# Autodesk Inventor assembly: 048-DXP(R,D-129)(F,D-166-3)
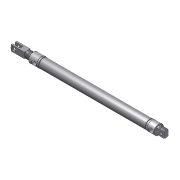
[picture p0: Inventor's stored thumbnail of the model, 180x180]
Saved by Autodesk Inventor 2012 (Build 160160000, 160)
## iProperties
Category: PARTsolutions
Created: 2013-01-19
Part Number: 048-DXP(R,D-129)(F,D-166-3)
Catalog Web Link: www.cadenas.de
Description: Original Line Standard Air Cylinders -
Document SubType Name: Assembly
Designer: PARTsolutions
NB: 048-DXP(R,D-129)(F,D-166-3)
NN: Original Line Standard Air Cylinders
NBSYN: $PNC.
LINA: 048-DXP
PSOL_MULTISOLIDPART: 0.0
PN: 048-DXP
PNC: 048-DXP(R,D-129)(F,D-166-3)
PNA: (D-129)(D-166-3)
DASH: -
BORE1: 0.75000000
BORE: 3/4" (04)
BOREPN: 04
STROKE: 8.000
STROKEALG: [0.011:50/0.001]
STROKE1: 8.000
ACTING: D
ACTINGALG: '' , 'Single Acting (SA)' , 'R' , 'Reverse Single Acting (SA)' , 'D' , 'Double Acting (SA)'
ACTINGPN: D
MNT: XP
MNTALG: '' , 'Front Nose Mounting (SA)' , 'P' , 'Rear Pivot Mounting (SA)' , 'XP' , 'Double End or Pivot Mounting (SA)' , 'X' , 'Double End Mounting (SA)' , 'BF' , 'Front Block Mounting (SA)' , 'BR' , 'Rear Block Mounting for Vertical Positioning (SA)' , 'BFT' , 'Front Block Trunnion Mounting (SA)' , 'BRT' , 'Rear Block Trunnion Mounting (SA)'
MNTPN: XP
DERALG: '' , 'N/A'
NRALG: '' , 'N/A'
BMALG: '' , 'N/A'
COALG: '' , 'N/A'
OOALG: '', 'N/A'
VO: Z
VOALG: 'Z' , 'N/A'
MALG: '', 'Without Magnet', 'M', 'With Magnet'
EEL: 0.000
EEMAX: 42.0000
EEALG: '', 'Without Extra Extension', 'EE', 'With Extra Extension'
EELALG: 0
EEPN1: 0.000
KALG: '', 'Standard' , 'K' , 'Ports Rotated 90deg K'
QALG: '' , 'N/A'
YALG: '' , 'Without Pivot Bushing' , 'Y' , 'With Pivot Bushing'
FALG: '', 'Non-Coated (Standard)', 'F', 'Molycoated'
TALG: '' , 'Standard -20° to 200°F (-29° to 95°C)' , 'N' , 'Low Temperature' , 'V' , 'High Temperature'
BALG: '', 'W/out Bumpers' , 'B' , 'W/ Bumpers'
HALG: '', 'N/A'
SERALG: '' , 'Without Spring Extend/Return' , 'JS' , 'With Spring Return' , 'JR' , 'With Spring Extend'
SRALG: '' , 'Standard Stainless Steel'
SRCON: 0
WALG: '' , 'Without Wiper' , 'W' , 'With Wiper'
EALG: '' , 'Standard Seals/Lube' , 'E' , 'Non-Lube Seals/Lube'
HLALG: '' , 'Without Low Pressure Hydraulic' , 'HL' , 'With Low Pressure Hydraulic'
STALG: '' , 'N/A'
STPT1ALG: '' , 'N/A'
STPT2ALG: '' , 'N/A'
STPT3ALG: '' , 'N/A'
STPT4ALG: '' , 'N/A'
MB: R,D-129
MBALG: '' , 'Without Mounting Bracket' , 'F,D-129' , 'D-129 (front)'  , 'R,D-129' , 'D-129 (rear)' , '2x,D-129' , 'D-129 (front & rear)'
MBPN: (R,D-129)
MBPNALL: D-129
MBPNALLREAR: D-129
PBALG: '' , 'N/A'
PBPNALL: D-13498-A
PRC: F,D-166-3
PRCALG: '' , 'W/out Pivot Rod Clevis' , 'F,D-166-3' , 'D-166-3 (front)'
PRCPN: (F,D-166-3)
PRCPNALL: D-166-3
TBALG: '' , 'N/A'
MNALG: '' , 'N/A'
TLEN: 9.2555
FRAC: 74.7500
RGDACCON: R
RHCON: P
RHCON1: P
RHCONON: 1
FNUTCON: 1
RNUTCON: 1
FNUTPN: D-9
RNUTPN: D-9
FNUTTRANS: 0.0000
RNUTTRANS: 0.0000
VHOLECON: 0
A1: 1.5940
A1N: 0.8750
A1P: 1.5940
A1B: 1.5940
A4: 0.2525
A4N: 0.3130
A4P: 0.2525
A5: 0.0300
A1H: 1.594
A1NH: 0.5310
A1PH: 1.5940
A1BH: 1.0940
A1SH: 1.2190
A2H: 0.2190
A2NH: 0.2190
LENGTH: 3.7500
LENGTH1: 3.7500
LENGTH2: 3.8100
MUL: 8.0000
MUL11: 8.0000
MUL22: 21.520
MUL33: 13.5200
MUL2: 8.0000
MUL211: 8.0000
MUL222: 2.6900
MUL233: 1.6900
SSS: 16.0000
RGLEN: 1.3715
RHLEN: 1.1230
SSS1: 9.0000
A13: 1.3120
DIF: 0.0000
G5: 0.6250
ON: 0
SSADD: 0.0000
BADD: 0.0000
MADD: 0.0000
NVADD: 0.0000
TRACKL: 8.9655
TRACKCON: D-74168
TRIMCON: 0
TRIMCON1: 0
PINCON: D-51
FSPACE: 0.8211
SPACE: 0.1286
TEXT: 0.2250
S1: 1.0000
D1: 0.8325
D1N: 0.8050
D1B: 0.8625
D1P: 0.8325
FA: 0.940
RA: 0.9400
PPATH: standard_air_cylinder_asmtpl.prj
MATALGHTML: <b>Standard Original Line:</b><dl><dt>Rod:</dt><dd>- Stainless Steel</dd><dd>&nbsp;&nbsp;(5/16 ? 9/16 Bores)</dd><dd>- High Strength Carbon Steel</dd><dd>&nbsp;&nbsp;(3/4 ? 3 Bore)</dd><dd>- Stainless Steel</dd><dd>&nbsp;&nbsp;(?X? style DXP/DX/DXDE?)</dd><dt>Bearings:</dt><dd>- Sintered Bronze</dd><dt>Body:</dt><dd>- 304 Stainless Steel</dd><dt>End Caps:</dt><dd>- Aluminum</dd><dt>Seals:</dt><dd>- Buna N</dd></dl>
ASSCFGPRA: 04DXP
MBPNA: (D-129)
PRCPNA: (D-166-3)
ASSOPTACC: STPT4
A: 11.75
HADD: 0.0000
WFL: 0.250
QADD: 0.000
QADD1: 0.440
TEST: 8.0000
STDNUTF: 1
STDNUTR: 1
KT: DUMMY
CreationOption_UseAsmMates: false
SUPPLIER: Bimba
ARTICLENO: 048-DXP(R,D-129)(F,D-166-3)
BOMINFO: 048-DXP
CREATOR: CADENAS GmbH
PSOL_IDENT_0: {\\10.0.0.242\data_v9\23d-libs\bimba\bimba\bimba_imperial\bimba_full_line\original_line_cylinders\st
PSOL_IDENT_1: andard_air_cylinders\standard_air_cylinder_asmtab.prj},325 {VTYP=3D},{STYP=ASSTAB},{NB=048-DXP(R,D-1
PSOL_IDENT_2: 29)(F,D-166-3)},{LINA=048-DXP},{NN=Original Line Standard Air Cylinders},{DATE=06.09.2012 11:26:56},
PSOL_IDENT_3: {GEOMDATE=06.09.2012},{VERSION=},{LINEID=50},{LINESUBID=-1},{WBVAR=STROKE,ACTING,MNT,DER,NR,BM,CO,OO
PSOL_IDENT_4: ,VO,M,EE,EEL,K,Q,Y,G,T,B,H,SER,SR,NT,W,HL,STPT1,STPT2,STPT3,STPT4,MB,PB,PRC,TB,MN}  {NB=048-DXP(R,D-
PSOL_IDENT_5: 129)(F,D-166-3)},{LINA=048-DXP},{KT=DUMMY},{PN=048-DXP},{PNC=048-DXP(R,D-129)(F,D-166-3)},{PNA=(D-12
PSOL_IDENT_6: 9)(D-166-3)},{DASH=-},{BORE1=0.75000000},{BORE=3/4\" (04)},{BOREPN=04},{STROKE=8.000},{STROKEALG=[0.
PSOL_IDENT_7: 011:50/0.001]},{STROKE1=8.000},{ACTING=D},{ACTINGALG= '' , 'Single Acting (SA)' , 'R' , 'Reverse Sin
PSOL_IDENT_8: gle Acting (SA)' , 'D' , 'Double Acting (SA)' },{ACTINGPN=D},{MNT=XP},{MNTALG= '' , 'Front Nose Moun
PSOL_IDENT_9: ting (SA)' , 'P' , 'Rear Pivot Mounting (SA)' , 'XP' , 'Double End or Pivot Mounting (SA)' , 'X' , '
PSOL_IDENT_10: Double End Mounting (SA)' , 'BF' , 'Front Block Mounting (SA)' , 'BR' , 'Rear Block Mounting for Ver
PSOL_IDENT_11: tical Positioning (SA)' , 'BFT' , 'Front Block Trunnion Mounting (SA)' , 'BRT' , 'Rear Block Trunnio
PSOL_IDENT_12: n Mounting (SA)' },{TYPE=},{MNTPN=XP},{DER=},{DERALG= '' , 'N/A' },{NR=},{NRALG= '' , 'N/A' },{NRPN=
PSOL_IDENT_13: },{BM=},{BMALG= '' , 'N/A' },{BMPN=},{CO=},{COALG= '' , 'N/A' },{OO=},{OOALG= '', 'N/A' },{OOPN=},{V
PSOL_IDENT_14: O=Z},{VOALG= 'Z' , 'N/A' },{VOPN=},{OOVOPN=},{M=},{MALG= '', 'Without Magnet', 'M', 'With Magnet' },
PSOL_IDENT_15: {EE=},{EEL=0.000},{EEMAX=42.0000},{EEALG= '', 'Without Extra Extension', 'EE', 'With Extra Extension
PSOL_IDENT_16: ' },{EELALG=0},{EEPN=},{EEPN1=0.000},{K=},{KALG= '', 'Standard' , 'K' , 'Ports Rotated 90deg K' },{K
PSOL_IDENT_17: PN=},{Q=},{QALG= '' , 'N/A' },{QPN=},{Y=},{YALG= '' , 'Without Pivot Bushing' , 'Y' , 'With Pivot Bu
PSOL_IDENT_18: shing' },{YPN=},{YCON=},{F=},{FALG= '', 'Non-Coated (Standard)', 'F', 'Molycoated' },{FPN=},{G=},{GP
PSOL_IDENT_19: N=},{GPN99=},{T=},{TALG= '' , 'Standard -20° to 200°F (-29° to 95°C)' , 'N' , 'Low Temperature' , 'V
PSOL_IDENT_20: ' , 'High Temperature' },{NPN=},{VPN=},{B=},{BALG= '', 'W/out Bumpers' , 'B' , 'W/ Bumpers' },{BPN=}
PSOL_IDENT_21: ,{H=},{HALG= '', 'N/A' },{HPN=},{SER=},{SERALG= '' , 'Without Spring Extend/Return' , 'JS' , 'With S
PSOL_IDENT_22: pring Return' , 'JR' , 'With Spring Extend' },{SR=},{SRALG= '' , 'Standard Stainless Steel' },{SRPN=
PSOL_IDENT_23: },{SRCON=0},{NT=},{NTPN=},{W=},{WALG= '' , 'Without Wiper' , 'W' , 'With Wiper' },{WPN=},{E=},{EALG=
PSOL_IDENT_24: '' , 'Standard Seals/Lube' , 'E' , 'Non-Lube Seals/Lube' },{EPN=},{HL=},{HLALG= '' , 'Without Low P
PSOL_IDENT_25: ressure Hydraulic' , 'HL' , 'With Low Pressure Hydraulic' },{ST=},{STALG= '' , 'N/A' },{STPT1=},{STP
PSOL_IDENT_26: T1ALG= '' , 'N/A' },{STPT2=},{STPT2ALG= '' , 'N/A' },{STPT3=},{STPT3ALG= '' , 'N/A' },{STPT4=},{STPT
PSOL_IDENT_27: 4ALG= '' , 'N/A' },{STPN=},{MB=R,D-129},{MBALG= '' , 'Without Mounting Bracket' , 'F,D-129' , 'D-129
PSOL_IDENT_28: (front)'  , 'R,D-129' , 'D-129 (rear)' , '2x,D-129' , 'D-129 (front & rear)'},{MBPN=(R,D-129)},{MBP
PSOL_IDENT_29: NALL=D-129},{MBPNALLREAR=D-129},{PB=},{PBALG= '' , 'N/A' },{PBPN=},{PBPNALL=D-13498-A},{PRC=F,D-166-
PSOL_IDENT_30: 3},{PRCALG= '' , 'W/out Pivot Rod Clevis' , 'F,D-166-3' , 'D-166-3 (front)' },{PRCPN=(F,D-166-3)},{P
PSOL_IDENT_31: RCPNALL=D-166-3},{TB=},{TBALG= '' , 'N/A' },{TBPN=},{TBPNALL=},{MN=},{MNALG= '' , 'N/A' },{MNPN=},{M
PSOL_IDENT_32: NCONF=},{MNCONR=},{TLEN=9.2555},{FRAC=74.7500},{RGCON=},{RGDACCON=R},{RHCON=P},{RHCON1=P},{RHCONON=1
PSOL_IDENT_33: },{RHACCON=},{FNUTCON=1},{RNUTCON=1},{FNUTPN=D-9},{RNUTPN=D-9},{FNUTTRANS=0.0000},{RNUTTRANS=0.0000}
PSOL_IDENT_34: ,{VHOLECON=0},{A1=1.5940},{A1N=0.8750},{A1P=1.5940},{A1B=1.5940},{A4=0.2525},{A4N=0.3130},{A4P=0.252
PSOL_IDENT_35: 5},{A5=0.0300},{A1H=1.594},{A1NH=0.5310},{A1PH=1.5940},{A1BH=1.0940},{A1SH=1.2190},{A2H=0.2190},{A2N
PSOL_IDENT_36: H=0.2190},{LENGTH=3.7500},{LENGTH1=3.7500},{LENGTH2=3.8100},{MUL=8.0000},{MUL11=8.0000},{MUL22=21.52
PSOL_IDENT_37: },{MUL33=13.5200},{MUL2=8.0000},{MUL211=8.0000},{MUL222=2.6900},{MUL233=1.6900},{SSS=16.0000},{RGLEN
PSOL_IDENT_38: =1.3715},{RHLEN=1.1230},{SSS1=9.0000},{A13=1.3120},{DIF=0.0000},{G5=0.6250},{ON=0},{SSADD=0.0000},{B
PSOL_IDENT_39: ADD=0.0000},{MADD=0.0000},{NVADD=0.0000},{TRACKL=8.9655},{TRACKCON=D-74168},{TRIMCON=0},{TRIMCON1=0}
PSOL_IDENT_40: ,{PINCON=D-51},{FSPACE=0.8211},{SPACE=0.1286},{TEXT=0.2250},{S1=1.0000},{D1=0.8325},{D1N=0.8050},{D1
PSOL_IDENT_41: B=0.8625},{D1P=0.8325},{FA=0.940},{RA=0.9400},{PPATH=standard_air_cylinder_asmtpl.prj},{MATALGHTML=<
PSOL_IDENT_42: b>Standard Original Line:</b><dl><dt>Rod:</dt><dd>- Stainless Steel</dd><dd>&nbsp;&nbsp;(5/16 ? 9/16
PSOL_IDENT_43: Bores)</dd><dd>- High Strength Carbon Steel</dd><dd>&nbsp;&nbsp;(3/4 ? 3 Bore)</dd><dd>- Stainless
PSOL_IDENT_44: Steel</dd><dd>&nbsp;&nbsp;(?X? style DXP/DX/DXDE?)</dd><dt>Bearings:</dt><dd>- Sintered Bronze</dd><
PSOL_IDENT_45: dt>Body:</dt><dd>- 304 Stainless Steel</dd><dt>End Caps:</dt><dd>- Aluminum</dd><dt>Seals:</dt><dd>-
PSOL_IDENT_46: Buna N</dd></dl>},{ASSCFGPRA=04DXP},{MBPNA=(D-129)},{MNPNA=},{PRCPNA=(D-166-3)},{ASSOPTACC=STPT4},{
PSOL_IDENT_47: A=11.75},{HADD=0.0000},{WFL=0.25},{QADD=0.000},{QADD1=0.440},{TEST=8.0000},{MNTB=},{STDNUTF=1},{STDN
PSOL_IDENT_48: UTR=1}
Title: 048-DXP
Author: Cadenas PARTsolutions
## Documents named in this file (7)
- Z:\UserData\Documents\Inventor\team1885frc\Pneumatics\048-DXP_8inStrokex075Bore\048_DXP_R_D_129__F_D_166_3_.iam
- Z:\UserData\Documents\Inventor\team1885frc\Pneumatics\048-DXP_8inStrokex075Bore\04R000_rod_guide.ipt
- Z:\UserData\Documents\Inventor\team1885frc\Pneumatics\048-DXP_8inStrokex075Bore\048_DXP0_rod.ipt
- Z:\UserData\Documents\Inventor\team1885frc\Pneumatics\048-DXP_8inStrokex075Bore\D_166_3_dummy.ipt
- Z:\UserData\Documents\Inventor\team1885frc\Pneumatics\048-DXP_8inStrokex075Bore\D_14055.ipt
- Z:\UserData\Documents\Inventor\team1885frc\Pneumatics\048-DXP_8inStrokex075Bore\04R_9_25550.ipt
- Z:\UserData\Documents\Inventor\team1885frc\Pneumatics\048-DXP_8inStrokex075Bore\04P0010_rear_head.ipt
## Components (6 placed, 6 different names)
1. 04R000_rod_guide:1 — Mate:1
2. D-166-3-dummy:1
3. 04R-9.25550:1
4. 04P0010_rear_head:1 — Mate:2
5. 048-DXP0_rod:1 — Mate:1, Mate:2, Mate:3, Mate:4
6. D-14055:1 — Mate:3, Mate:4
## Relationships (4: Mate 4)
- Mate:1: 04R000_rod_guide:1 ↔ 048-DXP0_rod:1
- Mate:2: 04P0010_rear_head:1 ↔ 048-DXP0_rod:1
- Mate:3: 048-DXP0_rod:1 ↔ D-14055:1
- Mate:4: 048-DXP0_rod:1 ↔ D-14055:1
